# Autodesk Inventor assembly: Sun_ToyTrainAssembly
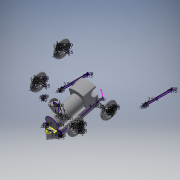
[picture p0: Inventor's stored thumbnail of the model, 180x180]
Saved by Autodesk Inventor 2016 (Build 200138000, 138)
## iProperties
Created: 2018-01-31
Part Number: Sun_ToyTrainAssembly
Document SubType Name: Assembly
Designer: Titus
Author: Titus
## Documents named in this file (8)
- E:\IED7_SunT\IED7_MouseTrap\Sun_ToyTrainAssembly.iam
- E:\IED7_SunT\IED7_ToyTrain\HitchPeg.ipt
- E:\IED7_SunT\IED7_ToyTrain\Sun_EngineBody.ipt
- E:\IED7_SunT\IED7_ToyTrain\Sun_Stack.ipt
- E:\IED7_SunT\IED7_ToyTrain\Sun_AxlePeg.ipt
- E:\IED7_SunT\IED7_ToyTrain\Sun_CowCatcher.ipt
- E:\IED7_SunT\IED7_ToyTrain\Sun_LinkageArm.ipt
- E:\IED7_SunT\IED7_ToyTrain\Sun_wheel.ipt
## Components (14 placed, 7 different names)
1. HitchPeg:1
2. Sun_EngineBody:1 — Mate:1, Mate:2, Mate:3, Mate:4, Mate:5, Mate:6, Mate:7, Mate:8, Mate:9, Mate:10, Mate:11, Mate:12, Mate:13, Mate:14, Mate:17, Mate:18, Mate:19
3. Sun_Stack:1 — Mate:1, Mate:5, Mate:6, Mate:14
4. Sun_AxlePeg:5 — Mate:20
5. Sun_AxlePeg:6 — Mate:21
6. Sun_AxlePeg:7 — Mate:8, Mate:16, Mate:17, Mate:18, Mate:19
7. Sun_AxlePeg:8 — Mate:7, Mate:9, Mate:10, Mate:11, Mate:12, Mate:13, Mate:15
8. Sun_CowCatcher:2 — Mate:2, Mate:3, Mate:4
9. Sun_LinkageArm:3
10. Sun_LinkageArm:4
11. Sun_wheel:1 — Mate:16
12. Sun_wheel:2 — Mate:20
13. Sun_wheel:3 — Mate:21
14. Sun_wheel:4 — Mate:15
## Relationships (21: Mate 21)
- Mate:1: Sun_EngineBody:1 ↔ Sun_Stack:1
- Mate:2: Sun_EngineBody:1 ↔ Sun_CowCatcher:2
- Mate:3: Sun_EngineBody:1 ↔ Sun_CowCatcher:2
- Mate:4: Sun_EngineBody:1 ↔ Sun_CowCatcher:2
- Mate:5: Sun_EngineBody:1 ↔ Sun_Stack:1
- Mate:6: Sun_EngineBody:1 ↔ Sun_Stack:1
- Mate:7: Sun_EngineBody:1 ↔ Sun_AxlePeg:8
- Mate:8: Sun_EngineBody:1 ↔ Sun_AxlePeg:7
- Mate:9: Sun_EngineBody:1 ↔ Sun_AxlePeg:8
- Mate:10: Sun_EngineBody:1 ↔ Sun_AxlePeg:8
- Mate:11: Sun_EngineBody:1 ↔ Sun_AxlePeg:8
- Mate:12: Sun_EngineBody:1 ↔ Sun_AxlePeg:8
- Mate:13: Sun_EngineBody:1 ↔ Sun_AxlePeg:8
- Mate:14: Sun_EngineBody:1 ↔ Sun_Stack:1
- Mate:15: Sun_AxlePeg:8 ↔ Sun_wheel:4
- Mate:16: Sun_AxlePeg:7 ↔ Sun_wheel:1
- Mate:17: Sun_EngineBody:1 ↔ Sun_AxlePeg:7
- Mate:18: Sun_EngineBody:1 ↔ Sun_AxlePeg:7
- Mate:19: Sun_EngineBody:1 ↔ Sun_AxlePeg:7
- Mate:20: Sun_AxlePeg:5 ↔ Sun_wheel:2
- Mate:21: Sun_AxlePeg:6 ↔ Sun_wheel:3
